# Autodesk Inventor assembly: Prototype Chasisi
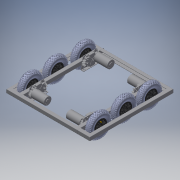
[picture p0: Inventor's stored thumbnail of the model, 180x180]
Saved by Autodesk Inventor 2016 (Build 200138000, 138)
## iProperties
Created: 2016-01-16
Part Number: Prototype Chasisi
Document SubType Name: Assembly
Designer: 17thorpc
Author: 17thorpc
## Documents named in this file (6)
- H:\2016 FRC CAD\Prototype Chasisi.iam
- H:\2016 FRC CAD\Chasis 28 piece.ipt
- H:\2016 FRC CAD\Chasis 28 piece front and back.ipt
- H:\2016 FRC CAD\Wheel 8.iam
- H:\2016 FRC CAD\CIMple Box A.iam
- H:\2016 FRC CAD\CIMple Box B.iam
## Components (16 placed, 5 different names)
1. Chasis 28 piece:1 — Mate:3, Mate:4, Flush:2, Flush:3, Flush:5, Mate:6, Flush:8, Flush:9
2. Chasis 28 piece:2 — Mate:1, Flush:1, Mate:2, Mate:3, Flush:3, Flush:5
3. Chasis 28 piece front and back:1 — Mate:1, Flush:1, Mate:2, Flush:4, Mate:5, Mate:7, Mate:17
4. Chasis 28 piece front and back:2 — Mate:4, Flush:2, Flush:4, Mate:5, Mate:6, Mate:7, Flush:6, Flush:7
5. Wheel 8:1 [sub-assembly] — Insert:2
6. Wheel 8:2 [sub-assembly] — Insert:4
7. Wheel 8:3 [sub-assembly] — Insert:3
8. Wheel 8:4 [sub-assembly]
9. Wheel 8:5 [sub-assembly] — Insert:1
10. Wheel 8:6 [sub-assembly]
11. Chasis 28 piece:3 — Flush:6, Mate:13, Mate:14, Mate:15, Mate:16, Mate:17
12. Chasis 28 piece:4 — Flush:7, Flush:8, Mate:9, Mate:10, Mate:11, Mate:12, Flush:9
13. CIMple Box A:1 [sub-assembly] — Mate:15, Mate:16, Insert:4
14. CIMple Box A:2 [sub-assembly] — Mate:11, Mate:12, Insert:2
15. CIMple Box B:1 [sub-assembly] — Mate:13, Mate:14, Insert:3
16. CIMple Box B:2 [sub-assembly] — Mate:9, Mate:10, Insert:1
## Relationships (29: Mate 16, Flush 9, Insert 4)
- Mate:1: Chasis 28 piece:2 ↔ Chasis 28 piece front and back:1
- Flush:1: Chasis 28 piece:2 ↔ Chasis 28 piece front and back:1
- Mate:2: Chasis 28 piece:2 ↔ Chasis 28 piece front and back:1
- Mate:3: Chasis 28 piece:1 ↔ Chasis 28 piece:2
- Mate:4: Chasis 28 piece:1 ↔ Chasis 28 piece front and back:2
- Flush:2: Chasis 28 piece:1 ↔ Chasis 28 piece front and back:2
- Flush:3: Chasis 28 piece:1 ↔ Chasis 28 piece:2
- Flush:4: Chasis 28 piece front and back:1 ↔ Chasis 28 piece front and back:2
- Mate:5: Chasis 28 piece front and back:1 ↔ Chasis 28 piece front and back:2
- Flush:5: Chasis 28 piece:1 ↔ Chasis 28 piece:2
- Mate:6: Chasis 28 piece:1 ↔ Chasis 28 piece front and back:2
- Mate:7: Chasis 28 piece front and back:1 ↔ Chasis 28 piece front and back:2
- Flush:6: Chasis 28 piece front and back:2 ↔ Chasis 28 piece:3
- Flush:7: Chasis 28 piece front and back:2 ↔ Chasis 28 piece:4
- Flush:8: Chasis 28 piece:1 ↔ Chasis 28 piece:4
- Mate:9 (-38.1 mm): Chasis 28 piece:4 ↔ CIMple Box B:2
- Mate:10: Chasis 28 piece:4 ↔ CIMple Box B:2
- Insert:1 (-44.45 mm): Wheel 8:5 ↔ CIMple Box B:2
- Mate:11 (-38.1 mm): Chasis 28 piece:4 ↔ CIMple Box A:2
- Mate:12: Chasis 28 piece:4 ↔ CIMple Box A:2
- Insert:2 (-6.35 mm): Wheel 8:1 ↔ CIMple Box A:2
- Mate:13 (-63.5 mm): Chasis 28 piece:3 ↔ CIMple Box B:1
- Mate:14: Chasis 28 piece:3 ↔ CIMple Box B:1
- Insert:3 (-9.525 mm): Wheel 8:3 ↔ CIMple Box B:1
- Mate:15 (-63.5 mm): Chasis 28 piece:3 ↔ CIMple Box A:1
- Mate:16: Chasis 28 piece:3 ↔ CIMple Box A:1
- Mate:17 (107.95 mm): Chasis 28 piece front and back:1 ↔ Chasis 28 piece:3
- Insert:4 (-9.525 mm): Wheel 8:2 ↔ CIMple Box A:1
- Flush:9 (-107.95 mm): Chasis 28 piece:1 ↔ Chasis 28 piece:4
